# Autodesk Inventor assembly: Assembly_Cube_Baseplate_4x1_v2
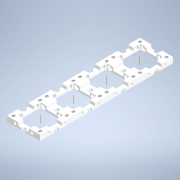
[picture p0: Inventor's stored thumbnail of the model, 180x180]
Saved by Autodesk Inventor 2022 (Build 260153000, 153)
## iProperties
Created: 2021-05-06
Part Number: Assembly_Cube_Baseplate_4x1_v2
Document SubType Name: Assembly
Designer: ASUS
Author: ASUS
## Documents named in this file (3)
- C:\Users\ASUS\Desktop\CAD designs\1. Crossed Polarizers\Assembly_Cube_Baseplate_4x1_v2.iam
- C:\Users\ASUS\Desktop\ASP - M.Sc. Photonics\Practical Modules\MODULE 3 - Research Project @IPHT-UC2\4.REF designing\10_Base_v0.ipt
- C:\Users\ASUS\Desktop\ASP - M.Sc. Photonics\Practical Modules\MODULE 3 - Research Project @IPHT-UC2\4.REF designing\00_BallMagnets_5mm.ipt
## Components (8 placed, 2 different names)
1. 10_Base_v0:1 — Rotational:1, Rigid:1
2. 10_Base_v0:2 — Rotational:1, Rotational:2, Rotational:3, Rigid:2
3. 10_Base_v0:3 — Rotational:2, Rotational:3, Rotational:4, Rotational:5, Rigid:3
4. 10_Base_v0:4 — Rotational:4, Rotational:5, Rigid:4
5. 00_BallMagnets_5mm:1 — Rigid:2
6. 00_BallMagnets_5mm:2 — Rigid:1
7. 00_BallMagnets_5mm:3 — Rigid:3
8. 00_BallMagnets_5mm:4 — Rigid:4
## Relationships (9: RevoluteJoint 5, WeldJoint 4)
- Rotational:1 [RevoluteJoint]: 10_Base_v0:1 ↔ 10_Base_v0:2
- Rotational:2 [RevoluteJoint]: 10_Base_v0:2 ↔ 10_Base_v0:3
- Rotational:3 [RevoluteJoint]: 10_Base_v0:2 ↔ 10_Base_v0:3
- Rotational:4 [RevoluteJoint]: 10_Base_v0:3 ↔ 10_Base_v0:4
- Rotational:5 [RevoluteJoint]: 10_Base_v0:3 ↔ 10_Base_v0:4
- Rigid:1 [WeldJoint] (2 mm): 10_Base_v0:1 ↔ 00_BallMagnets_5mm:2
- Rigid:2 [WeldJoint] (2 mm): 10_Base_v0:2 ↔ 00_BallMagnets_5mm:1
- Rigid:3 [WeldJoint] (2 mm): 10_Base_v0:3 ↔ 00_BallMagnets_5mm:3
- Rigid:4 [WeldJoint] (2 mm): 10_Base_v0:4 ↔ 00_BallMagnets_5mm:4
